# Autodesk Inventor assembly: ASY APN 1470 top funnel
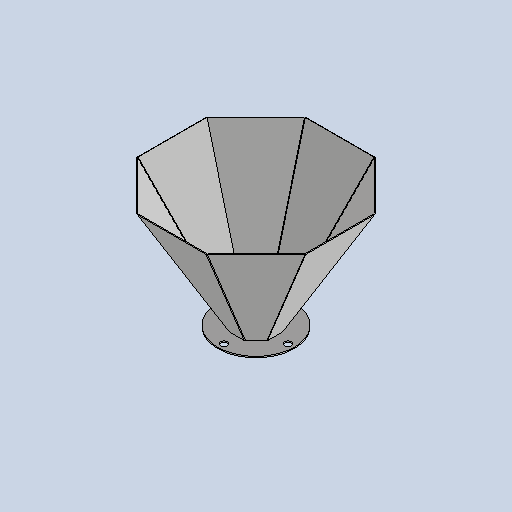
[picture p0: Inventor's stored thumbnail of the model, 512x512]
Saved by Autodesk Inventor 2025 (Build 290162010, 162A)
## iProperties
Created: 2025-07-11
Part Number: ASY APN 1470 top funnel
Document SubType Name: Assembly
Designer: user
Author: user
## Documents named in this file (3)
- C:\Users\admin\Yandex.Disk\home pc\Inventor\ANP-Antipayuta\ASY APN 1470 top funnel.iam
- C:\Users\admin\Yandex.Disk\home pc\Inventor\ANP-Antipayuta\APN 1471 top funnel wall.ipt
- C:\Users\admin\Yandex.Disk\home pc\Inventor\ANP-Antipayuta\APN 1472  funnel FLANGE 1200 50-90.ipt
## Components (3 placed, 2 different names)
1. APN 1472  funnel FLANGE 1200 50-90.ipt:1 — Mate:1, Mate:2, Mate:3, Mate:4, Mate:6, Mate:7
2. APN 1471 top funnel wall.ipt:1 — Mate:1, Mate:2, Mate:5, Mate:7
3. APN 1471 top funnel wall.ipt:2 — Mate:3, Mate:4, Mate:5, Mate:6
## Relationships (7: Mate 7)
- Mate:1: APN 1472  funnel FLANGE 1200 50-90.ipt:1 ↔ APN 1471 top funnel wall.ipt:1
- Mate:2: APN 1472  funnel FLANGE 1200 50-90.ipt:1 ↔ APN 1471 top funnel wall.ipt:1
- Mate:3: APN 1472  funnel FLANGE 1200 50-90.ipt:1 ↔ APN 1471 top funnel wall.ipt:2
- Mate:4: APN 1472  funnel FLANGE 1200 50-90.ipt:1 ↔ APN 1471 top funnel wall.ipt:2
- Mate:5: APN 1471 top funnel wall.ipt:1 ↔ APN 1471 top funnel wall.ipt:2
- Mate:6 (-2.87 mm): APN 1472  funnel FLANGE 1200 50-90.ipt:1 ↔ APN 1471 top funnel wall.ipt:2
- Mate:7 (-2.87 mm): APN 1472  funnel FLANGE 1200 50-90.ipt:1 ↔ APN 1471 top funnel wall.ipt:1
